# Autodesk Inventor assembly: M4-BallDevice
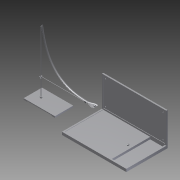
[picture p0: Inventor's stored thumbnail of the model, 180x180]
Saved by Autodesk Inventor 2012 SP2 (Build 160219200, 219)
## iProperties
Created: 2013-07-29
Part Number: M4-BallDevice
Document SubType Name: Assembly
Designer: 1
Author: 1
## Documents named in this file (5)
- D:\p3_metod1580library\figures\sources\M4-BallDevice\M4-BallDevice.iam
- D:\p3_metod1580library\figures\sources\M4-BallDevice\BallGuideAsmy.iam
- D:\p3_metod1580library\figures\sources\M4-BallDevice\CatcherBox.ipt
- D:\BoxCover.ipt
- D:\p3_metod1580library\figures\sources\M4-BallDevice\Ball.ipt
## Components (5 placed, 4 different names)
1. BallGuideAsmy:1 [sub-assembly] — Flush:1
2. CatcherBox:1 — Flush:5, Flush:6
3. BoxCover:1 — Flush:6
4. Ball:1
5. Ball:2
## Relationships (5: Flush 5)
- Flush:1: BallGuideAsmy:1
- [Flush]: BallGuideAsmy:1
- [Flush]: BallGuideAsmy:1
- Flush:5: CatcherBox:1
- Flush:6: CatcherBox:1 ↔ BoxCover:1
